# Autodesk Inventor assembly: ExtruderSatoer
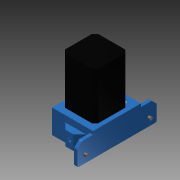
[picture p0: Inventor's stored thumbnail of the model, 180x180]
Saved by Autodesk Inventor 2015 SP1 (Build 190203100, 203)
## iProperties
Created: 2015-05-03
Part Number: ExtruderSatoer
Document SubType Name: Assembly
Designer: Jack
Author: Jack
## Documents named in this file (13)
- C:\Users\Jack\ownCloud\Projects\CrossBot\InventorModel\Extruder\ExtruderSatoer\ExtruderSatoer.iam
- C:\Users\Jack\ownCloud\Projects\CrossBot\InventorModel\Extruder\ExtruderSatoer\ExtruderSatoerBody.ipt
- C:\Users\Jack\ownCloud\Projects\CrossBot\InventorModel\Extruder\ExtruderSatoer\ExtruderSatoerMotorMount.ipt
- C:\Users\Jack\ownCloud\Projects\CrossBot\InventorModel\Hardware\Bolts\SHCS\SHCS4\SHCS4x30.ipt
- C:\Users\Jack\ownCloud\Projects\CrossBot\InventorModel\Extruder\ExtruderSatoer\ExtruderSatoerBearingArm.ipt
- C:\Users\Jack\ownCloud\Projects\CrossBot\InventorModel\Extruder\ExtruderSatoer\ExtruderSatoerCam.ipt
- C:\Users\Jack\ownCloud\Projects\CrossBot\InventorModel\Extruder\ExtruderSatoer\ExtruderSatoerCamArm.ipt
- C:\Users\Jack\ownCloud\Projects\CrossBot\InventorModel\Hardware\Bearing\BearingRadialBall\BearingRadialBall624zz.ipt
- C:\Users\Jack\ownCloud\Projects\CrossBot\InventorModel\Hardware\Bolts\SHCS\SHCS4\SHCS4x12.ipt
- C:\Users\Jack\ownCloud\Projects\CrossBot\InventorModel\Hardware\Nuts\Nut4.ipt
- C:\Users\Jack\ownCloud\Projects\CrossBot\InventorModel\Hardware\BoltWashers\BoltWasher4\BoltWasher4x8.iam
- C:\Users\Jack\ownCloud\Projects\CrossBot\InventorModel\Hardware\Bolts\SHCS\SHCS3\SHCS3x12.ipt
- C:\Users\Jack\ownCloud\Projects\CrossBot\InventorModel\Electronics\Motors\StepperMotorNema17x60mm.ipt
## Components (21 placed, 12 different names)
1. ExtruderSatoerBody:1 — Mate:4, Mate:5, Mate:6, Mate:7, Mate:8, Mate:9, Mate:13, Mate:15, Mate:16, Mate:22, Mate:23, Mate:24, Mate:25
2. ExtruderSatoerMotorMount:1 — Mate:29, Mate:30, Mate:31, Angle:2, Angle:3, Angle:4, Mate:32, Mate:33, Mate:34, Mate:35, Mate:36, Mate:37, Mate:38, Mate:39, Mate:40, Mate:42
3. SHCS4x30:1 — Mate:6, Mate:8, Mate:14, Mate:28
4. SHCS4x30:2 — Mate:5, Mate:7, Mate:12, Mate:26
5. SHCS4x30:3 — Mate:4, Mate:9, Mate:17, Mate:27
6. ExtruderSatoerBearingArm:1 — Mate:10, Mate:11, Mate:12, Mate:13, Mate:18, Mate:19, Angle:1, Mate:21
7. ExtruderSatoerCam:1 — Mate:16, Mate:17
8. ExtruderSatoerCamArm:1 — Mate:14, Mate:15
9. BearingRadialBall624zz:1 — Mate:10, Mate:11
10. SHCS4x12:1 — Mate:18, Mate:19, Mate:20
11. Nut4:1 — Mate:20, Angle:1, Mate:21
12. BoltWasher4x8:1 [sub-assembly] — Mate:22, Mate:25
13. BoltWasher4x8:2 [sub-assembly] — Mate:23, Mate:24
14. Nut4:2 — Mate:26, Mate:31, Angle:2
15. Nut4:3 — Mate:27, Mate:30, Angle:3
16. Nut4:4 — Mate:28, Mate:29, Angle:4
17. SHCS3x12:1 — Mate:34, Mate:37
18. SHCS3x12:2 — Mate:33, Mate:39
19. SHCS3x12:3 — Mate:35, Mate:36
20. SHCS3x12:4 — Mate:32, Mate:38, Mate:41
21. StepperMotorNema17x60mm:1 — Mate:40, Mate:41, Mate:42
## Relationships (46: Mate 42, Angle 4)
- [Mate] (0.25 mm): ExtruderSatoerBody:1 ↔ ExtruderSatoerMotorMount:1
- [Mate] (0.25 mm): ExtruderSatoerBody:1 ↔ ExtruderSatoerMotorMount:1
- [Mate]: ExtruderSatoerBody:1 ↔ ExtruderSatoerMotorMount:1
- Mate:4: ExtruderSatoerBody:1 ↔ SHCS4x30:3
- Mate:5: ExtruderSatoerBody:1 ↔ SHCS4x30:2
- Mate:6: ExtruderSatoerBody:1 ↔ SHCS4x30:1
- Mate:7: ExtruderSatoerBody:1 ↔ SHCS4x30:2
- Mate:8: ExtruderSatoerBody:1 ↔ SHCS4x30:1
- Mate:9: ExtruderSatoerBody:1 ↔ SHCS4x30:3
- Mate:10: ExtruderSatoerBearingArm:1 ↔ BearingRadialBall624zz:1
- Mate:11: ExtruderSatoerBearingArm:1 ↔ BearingRadialBall624zz:1
- Mate:12: SHCS4x30:2 ↔ ExtruderSatoerBearingArm:1
- Mate:13 (0.15 mm): ExtruderSatoerBody:1 ↔ ExtruderSatoerBearingArm:1
- Mate:14: SHCS4x30:1 ↔ ExtruderSatoerCamArm:1
- Mate:15 (0.15 mm): ExtruderSatoerBody:1 ↔ ExtruderSatoerCamArm:1
- Mate:16 (0.15 mm): ExtruderSatoerBody:1 ↔ ExtruderSatoerCam:1
- Mate:17: SHCS4x30:3 ↔ ExtruderSatoerCam:1
- Mate:18: ExtruderSatoerBearingArm:1 ↔ SHCS4x12:1
- Mate:19: ExtruderSatoerBearingArm:1 ↔ SHCS4x12:1
- Mate:20: SHCS4x12:1 ↔ Nut4:1
- Angle:1 (0 deg): ExtruderSatoerBearingArm:1 ↔ Nut4:1
- Mate:21: ExtruderSatoerBearingArm:1 ↔ Nut4:1
- Mate:22: ExtruderSatoerBody:1 ↔ BoltWasher4x8:1
- Mate:23: ExtruderSatoerBody:1 ↔ BoltWasher4x8:2
- Mate:24: ExtruderSatoerBody:1 ↔ BoltWasher4x8:2
- Mate:25: ExtruderSatoerBody:1 ↔ BoltWasher4x8:1
- Mate:26: SHCS4x30:2 ↔ Nut4:2
- Mate:27: SHCS4x30:3 ↔ Nut4:3
- Mate:28: SHCS4x30:1 ↔ Nut4:4
- Mate:29: ExtruderSatoerMotorMount:1 ↔ Nut4:4
- Mate:30: ExtruderSatoerMotorMount:1 ↔ Nut4:3
- Mate:31: ExtruderSatoerMotorMount:1 ↔ Nut4:2
- Angle:2 (0 deg): ExtruderSatoerMotorMount:1 ↔ Nut4:2
- Angle:3 (0 deg): ExtruderSatoerMotorMount:1 ↔ Nut4:3
- Angle:4 (0 deg): ExtruderSatoerMotorMount:1 ↔ Nut4:4
- Mate:32: ExtruderSatoerMotorMount:1 ↔ SHCS3x12:4
- Mate:33: ExtruderSatoerMotorMount:1 ↔ SHCS3x12:2
- Mate:34: ExtruderSatoerMotorMount:1 ↔ SHCS3x12:1
- Mate:35: ExtruderSatoerMotorMount:1 ↔ SHCS3x12:3
- Mate:36: ExtruderSatoerMotorMount:1 ↔ SHCS3x12:3
- Mate:37: ExtruderSatoerMotorMount:1 ↔ SHCS3x12:1
- Mate:38: ExtruderSatoerMotorMount:1 ↔ SHCS3x12:4
- Mate:39: ExtruderSatoerMotorMount:1 ↔ SHCS3x12:2
- Mate:40: ExtruderSatoerMotorMount:1 ↔ StepperMotorNema17x60mm:1
- Mate:41: SHCS3x12:4 ↔ StepperMotorNema17x60mm:1
- Mate:42: ExtruderSatoerMotorMount:1 ↔ StepperMotorNema17x60mm:1
